# Autodesk Inventor assembly: TKS 3000 Tarko Sale Bottom drain System
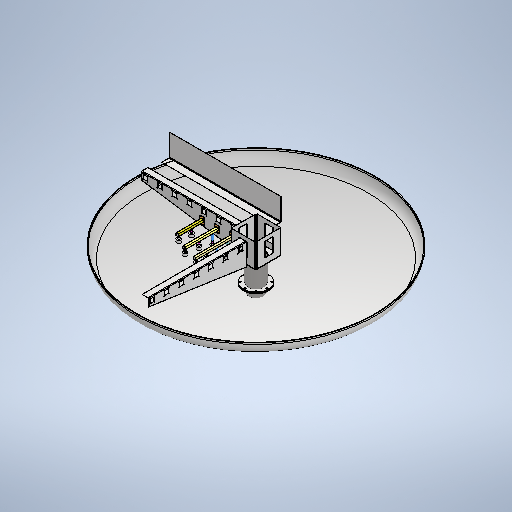
[picture p0: Inventor's stored thumbnail of the model, 512x512]
Saved by Autodesk Inventor 2025 (Build 290162010, 162A)
## iProperties
Created: 2025-07-14
Part Number: TKS 3000 Tarko Sale Bottom drain System
Document SubType Name: Assembly
Designer: user
Author: user
## Documents named in this file (18)
- C:\Users\admin\Yandex.Disk\home pc\Inventor\TKS-Tarko Sale\TKS 3000 Tarko Sale Bottom drain System.iam
- C:\Users\admin\Yandex.Disk\home pc\Inventor\TKS-Tarko Sale\dished head.ipt
- C:\Users\admin\Yandex.Disk\home pc\Inventor\TKS-Tarko Sale\DSB 111 outer tube.ipt
- C:\Users\admin\Yandex.Disk\home pc\Inventor\TKS-Tarko Sale\Main filter Flange.ipt
- C:\Users\admin\Yandex.Disk\home pc\Inventor\TKS-Tarko Sale\000 DSB dimentions.ipt
- C:\Users\admin\Yandex.Disk\home pc\Inventor\TKS-Tarko Sale\TKS 3001 BOTTOM DS main flange.ipt
- C:\Users\admin\Yandex.Disk\home pc\Inventor\TKS-Tarko Sale\TKS 3002 BOTTOM DS main tube.ipt
- C:\Users\admin\Yandex.Disk\home pc\Inventor\TKS-Tarko Sale\TKS 3003 BOTTOM DS reduce flange.ipt
- C:\Users\admin\Yandex.Disk\home pc\Inventor\TKS-Tarko Sale\TKS 3004 BOTTOM DS box wall 1.ipt
- C:\Users\admin\Yandex.Disk\home pc\Inventor\TKS-Tarko Sale\TKS 3005 BOTTOM DS diameter way.ipt
- C:\Users\admin\Yandex.Disk\home pc\Inventor\TKS-Tarko Sale\TKS 3006 BOTTOM DS diameter way blind.ipt
- C:\Users\admin\Yandex.Disk\home pc\Inventor\TKS-Tarko Sale\BOTTOM DS\ASY PNS 1752 FDS way 2.iam
- C:\Users\admin\Yandex.Disk\home pc\Inventor\TKS-Tarko Sale\BOTTOM DS\ASY PNS FDS way1.iam
- C:\Users\admin\Yandex.Disk\home pc\Inventor\TKS-Tarko Sale\BOTTOM DS\ASY PNS FDS way3.iam
- C:\Users\admin\Yandex.Disk\home pc\Inventor\TKS-Tarko Sale\TKS 3102 TOP DS main tube.ipt
- C:\Users\admin\Yandex.Disk\home pc\Inventor\TKS-Tarko Sale\TKS 3103 TOP DS outer tube.ipt
- C:\Users\admin\Yandex.Disk\home pc\Inventor\TKS-Tarko Sale\TKS 3109 top DS main flange.ipt
- C:\Users\admin\Yandex.Disk\home pc\Inventor\TKS-Tarko Sale\TKS 3108 top DS double flange.ipt
## Components (22 placed, 19 different names)
1. dished head.ipt:1 — Flush:2, Mate:1, Flush:3, Rigid:1
2. DSB 111 outer tube.ipt:1 — Rigid:1, Rigid:2
3. Main filter Flange.ipt:1 — Rigid:2, Rigid:3, Rigid:4
4. 000 DSB dimentions.ipt:1
5. TKS 3001 BOTTOM DS main flange:1 — Rigid:3
6. TKS 3002 BOTTOM DS main tube:1 — Rigid:4, Rigid:5
7. TKS 3003 BOTTOM DS reduce flange:1 — Rigid:5, Rigid:6, Rigid:7
8. TKS 3004 BOTTOM DS box wall 1:1 — Rigid:6, Rigid:16, Rigid:17
9. TKS 3004 BOTTOM DS box wall 1:2 — Rigid:7
10. TKS 3005 BOTTOM DS diameter way:1 — Rigid:16
11. TKS 3006 BOTTOM DS diameter way blind:1
12. ASY PNS 1752 FDS way 2:1 [sub-assembly]
13. ASY PNS FDS way1:1 [sub-assembly]
14. ASY PNS FDS way3:1 [sub-assembly]
15. TKS 3102 TOP DS main tube:1 — Rotational:1
16. TKS 3103 TOP DS outer tube:1 — Rigid:14
17. TKS 3001 BOTTOM DS main flange:2 — Rigid:13
18. TKS 3109 top DS main flange:1 — Rotational:1, Rigid:15, Rotational:2
19. DSB 111 outer tube:2 — Rigid:13, Rotational:2, Rotational:3
20. TKS 3108 top DS double flange:1 — Rigid:14, Rigid:15
21. dished head:2 — Rotational:3
22. TKS 3005 BOTTOM DS diameter way:2 — Rigid:17
## Relationships (18: WeldJoint 12, RevoluteJoint 3, Flush 2, Mate 1)
- Flush:2: dished head.ipt:1
- Mate:1: dished head.ipt:1
- Flush:3: dished head.ipt:1
- Rigid:1 [WeldJoint]: dished head.ipt:1 ↔ DSB 111 outer tube.ipt:1
- Rigid:2 [WeldJoint]: DSB 111 outer tube.ipt:1 ↔ Main filter Flange.ipt:1
- Rigid:3 [WeldJoint]: Main filter Flange.ipt:1 ↔ TKS 3001 BOTTOM DS main flange:1
- Rigid:4 [WeldJoint]: Main filter Flange.ipt:1 ↔ TKS 3002 BOTTOM DS main tube:1
- Rigid:5 [WeldJoint]: TKS 3002 BOTTOM DS main tube:1 ↔ TKS 3003 BOTTOM DS reduce flange:1
- Rigid:6 [WeldJoint]: TKS 3003 BOTTOM DS reduce flange:1 ↔ TKS 3004 BOTTOM DS box wall 1:1
- Rigid:7 [WeldJoint]: TKS 3003 BOTTOM DS reduce flange:1 ↔ TKS 3004 BOTTOM DS box wall 1:2
- Rigid:13 [WeldJoint]: TKS 3001 BOTTOM DS main flange:2 ↔ DSB 111 outer tube:2
- Rotational:1 [RevoluteJoint]: TKS 3102 TOP DS main tube:1 ↔ TKS 3109 top DS main flange:1
- Rigid:14 [WeldJoint]: TKS 3103 TOP DS outer tube:1 ↔ TKS 3108 top DS double flange:1
- Rigid:15 [WeldJoint]: TKS 3109 top DS main flange:1 ↔ TKS 3108 top DS double flange:1
- Rotational:2 [RevoluteJoint]: TKS 3109 top DS main flange:1 ↔ DSB 111 outer tube:2
- Rotational:3 [RevoluteJoint]: DSB 111 outer tube:2 ↔ dished head:2
- Rigid:16 [WeldJoint]: TKS 3004 BOTTOM DS box wall 1:1 ↔ TKS 3005 BOTTOM DS diameter way:1
- Rigid:17 [WeldJoint]: TKS 3004 BOTTOM DS box wall 1:1 ↔ TKS 3005 BOTTOM DS diameter way:2
